# Autodesk Inventor assembly: 2 Falcon Single Reduction (WCP-0234)
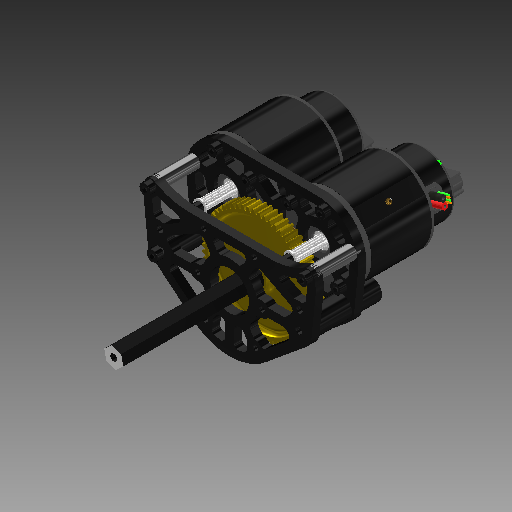
[picture p0: Inventor's stored thumbnail of the model, 512x512]
Saved by Autodesk Inventor 2023 (Build 270158000, 158)
## iProperties
Created: 2019-12-21
Part Number: 2 Falcon Single Reduction (WCP-0234)
Description: STEP AP214
Document SubType Name: Assembly
Designer: Desktop
Sending System: SolidWorks 2018
Preprocessor: SwSTEP 2.0
Title: WCP-0234 Rev1 - WCP SS Gearbox (Single Speed, 1 Stage).STEP
Revision Number: ANY
## iProperties of the stored document MemberDocs/xLqvepmqnB0sscau4Ttppawfh5h
Created: 2019-12-21
Part Number: 2 Falcon Single Reduction (WCP-0234)
Description: STEP AP214
Document SubType Name: Assembly
Designer: Desktop
Sending System: SolidWorks 2018
Preprocessor: SwSTEP 2.0
Title: WCP-0234 Rev1 - WCP SS Gearbox (Single Speed, 1 Stage).STEP
Revision Number: ANY
## iProperties of the stored document MemberDocs/x1zyynaqtFcftaj5mKokjps2x2f
Created: 2019-12-21
Part Number: 2 Falcon Single Reduction (WCP-0234)
Description: STEP AP214
Document SubType Name: Assembly
Designer: Desktop
Sending System: SolidWorks 2018
Preprocessor: SwSTEP 2.0
Title: WCP-0234 Rev1 - WCP SS Gearbox (Single Speed, 1 Stage).STEP
Revision Number: ANY
## iProperties of the stored document MemberDocs/xMxjli5cnGc0axyes40ohqydbMd
Created: 2019-12-21
Part Number: 2 Falcon Single Reduction (WCP-0234)
Description: STEP AP214
Document SubType Name: Assembly
Designer: Desktop
Sending System: SolidWorks 2018
Preprocessor: SwSTEP 2.0
Title: WCP-0234 Rev1 - WCP SS Gearbox (Single Speed, 1 Stage).STEP
Revision Number: ANY
## iProperties of the stored document MemberDocs/xPnixdcmtAsxrbsslCladjitsFg
Created: 2019-12-21
Part Number: 2 Falcon Single Reduction (WCP-0234)
Description: STEP AP214
Document SubType Name: Assembly
Designer: Desktop
Sending System: SolidWorks 2018
Preprocessor: SwSTEP 2.0
Title: WCP-0234 Rev1 - WCP SS Gearbox (Single Speed, 1 Stage).STEP
Revision Number: ANY
## Documents named in this file (62)
- C:\Users\Cal\Desktop\Robotics\Design\Collaborative\Collaborative Parts Library\Drivetrains\COTS WCD Gearboxes\2 Falcon Single Reduction (WCP-0234).iam
- C:\Users\Cal\Desktop\Robotics\Design\Collaborative\Collaborative Parts Library\Drivetrains\COTS WCD Gearboxes\2 Falcon Single Reduction (WCP-0234)\WCP-0234-001 Rev1.ipt
- C:\Users\Cal\Desktop\Robotics\Design\Collaborative\Collaborative Parts Library\Drivetrains\COTS WCD Gearboxes\2 Falcon Single Reduction (WCP-0234)\WCP-0234-002 Rev1.ipt
- C:\Users\Cal\Desktop\Robotics\Design\Collaborative\Collaborative Parts Library\Drivetrains\VersaChassis Parts\217-3437.ipt
- C:\Users\Cal\Desktop\Robotics\Design\Collaborative\Collaborative Parts Library\Power Transfer\Bearings and Bushings\Bearings\FR8 Hex.ipt
- E:\Middleton Robotics\Collaborative Robots\Collaborative Part Library\Power Transfer\Bearings.ipt
- C:\Users\Cal\Desktop\Robotics\Design\Collaborative\Collaborative Parts Library\Shaft Retention\Snaprings\Snapring for 0.5in Shaft (0.461in).ipt
- E:\Middleton Robotics\Collaborative Robots\Collaborative Part Library\Shaft Retention\Snaprings.ipt
- E:\Middleton Robotics\Collaborative Robots\Collaborative Part Library\Hardware\Machine Screws.ipt
- C:\Users\Cal\Desktop\Robotics\Design\Collaborative\Collaborative Parts Library\Hardware\Fasteners\Machine Screws\10-32 UNFx0.75 Socket Head Cap Screw.ipt
- E:\Middleton Robotics\Collaborative Robots\Collaborative Part Library\Hardware\Nuts.ipt
- C:\Users\Cal\Desktop\Robotics\Design\Collaborative\Collaborative Parts Library\Hardware\Nuts and Threaded Blocks\Nuts\10-32 Pan Head Nylon locknut.ipt
- C:\Users\Cal\Desktop\Robotics\Design\Collaborative\Collaborative Parts Library\Hardware\Fasteners\Machine Screws\10-32 UNFx0.25 Button Head Cap Screw.ipt
- C:\Users\Cal\Desktop\Robotics\Design\Collaborative\Collaborative Parts Library\Motors\FRC\Falcon 500.ipt
- C:\Users\Cal\Desktop\Robotics\Design\Collaborative\Collaborative Parts Library\Drivetrains\COTS WCD Gearboxes\2 Falcon Single Reduction (WCP-0234)\WCP-0234-003 Rev1.ipt
- C:\Users\Cal\Desktop\Robotics\Design\Collaborative\Collaborative Parts Library\Hardware\Fasteners\Machine Screws.ipt
- C:\Users\Cal\Desktop\Robotics\Design\Collaborative\Collaborative Parts Library\Hardware\Spacers\Spacers & Standoffs.ipt
- C:\Users\Cal\Desktop\Robotics\Design\Collaborative\Collaborative Parts Library\Hardware\Spacers\Spacers & Standoffs\WCP Aluminum Standoff (No. 10 x 1Lg x 0.375OD).ipt
- C:\Users\Cal\Desktop\Robotics\Design\Collaborative\Collaborative Parts Library\Hardware\Spacers\Spacers & Standoffs\Nylon Unthreaded Spacer (No. 10 x 1.25Lg x 0.625OD).ipt
- C:\Users\Cal\Desktop\Robotics\Design\Collaborative\Collaborative Parts Library\Motors\FRC\Motor Pinions.ipt
- C:\Users\Cal\Desktop\Robotics\Design\Collaborative\Collaborative Parts Library\Hardware\Fasteners\Machine Screws\8-32 UNCx0.25 Socket Head Cap Screw.ipt
- C:\Users\Cal\Desktop\Robotics\Design\Collaborative\Collaborative Parts Library\Hardware\Fasteners\Washers\Washer 0.174ID 0.375OD 0.038Thick.ipt
- E:\Middleton Robotics\Collaborative Robots\Collaborative Part Library\Hardware\Fasteners\Washers.ipt
- C:\Users\Cal\Desktop\Robotics\Design\Collaborative\Collaborative Parts Library\Power Transfer\Gears (Hex)\VexPro Spur Gears.ipt
- C:\Users\Cal\Desktop\Robotics\Design\Collaborative\Collaborative Parts Library\Hardware\Fasteners\Machine Screws\10-32 UNFx1.75 Socket Head Cap Screw.ipt
- C:\Users\Cal\Desktop\Robotics\Design\Collaborative\Collaborative Parts Library\Hardware\Fasteners\Machine Screws\10-32 UNFx2 Socket Head Cap Screw.ipt
- C:\Users\Cal\Desktop\Robotics\Design\Collaborative\Collaborative Parts Library\Power Transfer\Gears (Hex)\Spur Gear2\20dp 62T VexPro 500 Hex Aluminum Gear (Pocketed).ipt
- C:\Users\Cal\Desktop\Robotics\Design\Collaborative\Collaborative Parts Library\Hardware\Spacers\Spacers & Standoffs\WCP Aluminum Standoff (No. 10 x 1.25Lg x 0.375OD).ipt
- C:\Users\Cal\Desktop\Robotics\Design\Collaborative\Collaborative Parts Library\Hardware\Fasteners\Machine Screws\10-32 UNFx1.125 Socket Head Cap Screw.ipt
- E:\Middleton Robotics\Collaborative Robots\Collaborative Part Library\Drivetrains\COTS WCD Gearboxes\2 Falcon Single Reduction (WCP-0234)\WCP-0234-001 Rev1.ipt
- E:\Middleton Robotics\Collaborative Robots\Collaborative Part Library\Drivetrains\COTS WCD Gearboxes\2 Falcon Single Reduction (WCP-0234)\WCP-0234-002 Rev1.ipt
- E:\Middleton Robotics\Collaborative Robots\Collaborative Part Library\Drivetrains\217-3437.ipt
- E:\Middleton Robotics\Collaborative Robots\Collaborative Part Library\Power Transfer\Bearings and Bushings\Bearings\FR8 Hex.ipt
- E:\Middleton Robotics\Collaborative Robots\Collaborative Part Library\Shaft Retention\Snaprings\Snapring for 0.5in Shaft (0.461in).ipt
- E:\Middleton Robotics\Collaborative Robots\Collaborative Part Library\Hardware\Fasteners\Machine Screws\10-32 UNFx0.75 Socket Head Cap Screw.ipt
- E:\Middleton Robotics\Collaborative Robots\Collaborative Part Library\Hardware\Nuts and Threaded Blocks\Nuts\10-32 Pan Head Nylon locknut.ipt
- E:\Middleton Robotics\Collaborative Robots\Collaborative Part Library\Hardware\Fasteners\Machine Screws\10-32 UNFx0.25 Button Head Cap Screw.ipt
- E:\Middleton Robotics\Collaborative Robots\Collaborative Part Library\Motors\FRC\Falcon 500.ipt
- E:\Middleton Robotics\Collaborative Robots\Collaborative Part Library\Drivetrains\COTS WCD Gearboxes\2 Falcon Single Reduction (WCP-0234)\WCP-0234-003 Rev1.ipt
- E:\Middleton Robotics\Collaborative Robots\Collaborative Part Library\Hardware\Fasteners\Machine Screws.ipt
- E:\Middleton Robotics\Collaborative Robots\Collaborative Part Library\Hardware\Spacers\Spacers & Standoffs.ipt
- E:\Middleton Robotics\Collaborative Robots\Collaborative Part Library\Hardware\Spacers\Spacers & Standoffs\WCP Aluminum Standoff (No. 10 x 1Lg x 0.375OD).ipt
- E:\Middleton Robotics\Collaborative Robots\Collaborative Part Library\Hardware\Spacers\Spacers & Standoffs\Nylon Unthreaded Spacer (No. 10 x 1.25Lg x 0.625OD).ipt
- E:\Middleton Robotics\Collaborative Robots\Collaborative Part Library\Motors\FRC\Motor Pinions.ipt
- E:\Middleton Robotics\Collaborative Robots\Collaborative Part Library\Hardware\Fasteners\Machine Screws\8-32 UNCx0.25 Socket Head Cap Screw.ipt
- E:\Middleton Robotics\Collaborative Robots\Collaborative Part Library\Hardware\Fasteners\Washers\Washer 0.174ID 0.375OD 0.038Thick.ipt
- E:\Middleton Robotics\Collaborative Robots\Collaborative Part Library\Power Transfer\Gears (Hex)\VexPro Spur Gears.ipt
- E:\Middleton Robotics\Collaborative Robots\Collaborative Part Library\Hardware\Fasteners\Machine Screws\10-32 UNFx1.75 Socket Head Cap Screw.ipt
- E:\Middleton Robotics\Collaborative Robots\Collaborative Part Library\Hardware\Fasteners\Machine Screws\10-32 UNFx2 Socket Head Cap Screw.ipt
- E:\Middleton Robotics\Collaborative Robots\Collaborative Part Library\Power Transfer\Gears (Hex)\Spur Gear2\20dp 62T VexPro 500 Hex Aluminum Gear (Pocketed).ipt
- E:\Middleton Robotics\Collaborative Robots\Collaborative Part Library\Power Transfer\Gears (Hex)\Spur Gear2\20dp 58T VexPro 500 Hex Aluminum Gear (Pocketed).ipt
- E:\Middleton Robotics\Collaborative Robots\Collaborative Part Library\Power Transfer\VexPro Spur Gears.ipt
- E:\Middleton Robotics\Collaborative Robots\Collaborative Part Library\Drivetrains\VersaWheel Configurator.iam
- E:\Middleton Robotics\Collaborative Robots\Collaborative Part Library\Power Transfer\Sprockets\VexPro Sprockets.ipt
- E:\Middleton Robotics\Collaborative Robots\Collaborative Part Library\Power Transfer\Bearing Blocks\VersaBlock V2 (217-6111).ipt
- E:\Middleton Robotics\Collaborative Robots\Collaborative Part Library\Hardware\Fasteners\Washers\Washer 0.265ID 0.688OD 0.055Thick.ipt
- E:\Middleton Robotics\Collaborative Robots\Collaborative Part Library\Hardware\Retention\Washers.ipt
- E:\Middleton Robotics\Collaborative Robots\Collaborative Part Library\Hardware\Fasteners\Machine Screws\1(_FS)4-20 UNCx0.5 Button Head Cap Screw.ipt
- E:\Middleton Robotics\Collaborative Robots\Collaborative Part Library\Hardware\Fasteners\Machine Screws\10-32 UNFx1.5 Socket Head Cap Screw.ipt
- E:\Middleton Robotics\Collaborative Robots\Collaborative Part Library\Power Transfer\Sprockets\Sprockets\VexPro 12T 35 Chain 500 Hex Bore Double Sprocket.ipt
- E:\Middleton Robotics\Collaborative Robots\Collaborative Part Library\Hardware\Spacers\Spacers & Standoffs\WCP Aluminum Standoff (No. 10 x 1.75Lg x 0.375OD).ipt
- E:\Middleton Robotics\Collaborative Robots\Collaborative Part Library\Hardware\Fasteners\Machine Screws\10-32 UNFx2.5 Socket Head Cap Screw.ipt
## Components (35 placed, 20 different names)
1. WCP-0234-001 Rev1_1 — Insert:3, Mate:1, Mate:2, Insert:17, Insert:18, Insert:19, Insert:20, Insert:21, Insert:22, Insert:23, Insert:24, Insert:25, Insert:26, Insert:27, Flush:1, Insert:45, Insert:48
2. WCP-0234-002 Rev1_2 — Insert:6, Insert:7, Insert:13, Insert:14, Insert:15, Insert:16, Insert:32, Insert:33, Flush:2, Insert:42, Insert:44, Flush:3
3. 20dp 62T VexPro 500 Hex Aluminum Gear (Pocketed):1 — Insert:5
4. 217-3437:1 — Insert:4, Insert:12, Mate:6
5. FR8 Hex:1 — Insert:3, Insert:4, Insert:5
6. WCP Aluminum Standoff (No. 10 x 1.25Lg x 0.375OD):5 — Insert:7, Mate:2
7. WCP Aluminum Standoff (No. 10 x 1.25Lg x 0.375OD):4 — Insert:6, Mate:1, Insert:45, Insert:48
8. Snapring for 0.5in Shaft (0.461in):1 — Insert:12
9. 10-32 UNFx2 Socket Head Cap Screw:23 — Insert:14
10. 10-32 UNFx2 Socket Head Cap Screw:22 — Insert:13
11. 10-32 UNFx1.125 Socket Head Cap Screw:19 — Insert:16
12. 10-32 UNFx1.75 Socket Head Cap Screw:21 — Insert:15
13. 10-32 UNFx0.75 Socket Head Cap Screw:5 — Insert:18
14. 10-32 UNFx0.75 Socket Head Cap Screw:6 — Insert:17, Mate:4
15. 10-32 UNFx0.75 Socket Head Cap Screw:7 — Insert:19
16. 10-32 UNFx0.75 Socket Head Cap Screw:8 — Insert:21
17. 10-32 UNFx0.75 Socket Head Cap Screw:9 — Insert:22
18. 10-32 UNFx0.75 Socket Head Cap Screw:10 — Insert:20, Mate:5
19. 10-32 Pan Head Nylon locknut:1 — Insert:23
20. 10-32 Pan Head Nylon locknut:3 — Insert:24
21. Falcon 500:1 — Insert:26, Mate:5, Insert:49, Insert:52
22. Falcon 500:2 — Insert:27, Mate:4, Insert:50, Insert:54
23. WCP-0234-003 Rev1:1 — Insert:33
24. WCP-0234-003 Rev1:2 — Insert:32
25. WCP Aluminum Standoff (No. 10 x 1Lg x 0.375OD):10 — Insert:42
26. Nylon Unthreaded Spacer (No. 10 x 1.25Lg x 0.625OD):12 — Insert:44
27. Motor Pinions:1 — Insert:49
28. Motor Pinions:2 — Insert:50
29. 8-32 UNCx0.25 Socket Head Cap Screw:32 — Insert:51
30. Washer 0.174ID 0.375OD 0.038Thick:2 — Insert:51, Insert:52
31. 8-32 UNCx0.25 Socket Head Cap Screw:36
32. Washer 0.174ID 0.375OD 0.038Thick:3 — Insert:54
33. 10-32 UNFx0.25 Button Head Cap Screw:11 — Insert:25
34. 10-32 UNFx0.25 Button Head Cap Screw:12
35. 10-32 UNFx0.25 Button Head Cap Screw:13
## Component patterns: (3 elements, first: 10-32 UNFx0.25 Button Head Cap Screw:11)
## Relationships (41: Insert 33, Mate 5, Flush 3)
- Insert:3: WCP-0234-001 Rev1_1 ↔ FR8 Hex:1
- Insert:4: 217-3437:1 ↔ FR8 Hex:1
- Insert:5: 20dp 62T VexPro 500 Hex Aluminum Gear (Pocketed):1 ↔ FR8 Hex:1
- Insert:6: WCP-0234-002 Rev1_2 ↔ WCP Aluminum Standoff (No. 10 x 1.25Lg x 0.375OD):4
- Insert:7: WCP-0234-002 Rev1_2 ↔ WCP Aluminum Standoff (No. 10 x 1.25Lg x 0.375OD):5
- Mate:1: WCP-0234-001 Rev1_1 ↔ WCP Aluminum Standoff (No. 10 x 1.25Lg x 0.375OD):4
- Mate:2: WCP-0234-001 Rev1_1 ↔ WCP Aluminum Standoff (No. 10 x 1.25Lg x 0.375OD):5
- Insert:12: 217-3437:1 ↔ Snapring for 0.5in Shaft (0.461in):1
- Insert:13: WCP-0234-002 Rev1_2 ↔ 10-32 UNFx2 Socket Head Cap Screw:22
- Insert:14: WCP-0234-002 Rev1_2 ↔ 10-32 UNFx2 Socket Head Cap Screw:23
- Insert:15 (1.5875 mm): WCP-0234-002 Rev1_2 ↔ 10-32 UNFx1.75 Socket Head Cap Screw:21
- Insert:16 (1.5875 mm): WCP-0234-002 Rev1_2 ↔ 10-32 UNFx1.125 Socket Head Cap Screw:19
- Insert:17: WCP-0234-001 Rev1_1 ↔ 10-32 UNFx0.75 Socket Head Cap Screw:6
- Insert:18: WCP-0234-001 Rev1_1 ↔ 10-32 UNFx0.75 Socket Head Cap Screw:5
- Insert:19: WCP-0234-001 Rev1_1 ↔ 10-32 UNFx0.75 Socket Head Cap Screw:7
- Insert:20: WCP-0234-001 Rev1_1 ↔ 10-32 UNFx0.75 Socket Head Cap Screw:10
- Insert:21: WCP-0234-001 Rev1_1 ↔ 10-32 UNFx0.75 Socket Head Cap Screw:8
- Insert:22: WCP-0234-001 Rev1_1 ↔ 10-32 UNFx0.75 Socket Head Cap Screw:9
- Insert:23: WCP-0234-001 Rev1_1 ↔ 10-32 Pan Head Nylon locknut:1
- Insert:24: WCP-0234-001 Rev1_1 ↔ 10-32 Pan Head Nylon locknut:3
- Insert:25 (1.5875 mm): WCP-0234-001 Rev1_1 ↔ 10-32 UNFx0.25 Button Head Cap Screw:11
- Insert:26: WCP-0234-001 Rev1_1 ↔ Falcon 500:1
- Insert:27: WCP-0234-001 Rev1_1 ↔ Falcon 500:2
- Mate:4: 10-32 UNFx0.75 Socket Head Cap Screw:6 ↔ Falcon 500:2
- Mate:5: 10-32 UNFx0.75 Socket Head Cap Screw:10 ↔ Falcon 500:1
- Insert:32: WCP-0234-002 Rev1_2 ↔ WCP-0234-003 Rev1:2
- Insert:33: WCP-0234-002 Rev1_2 ↔ WCP-0234-003 Rev1:1
- Mate:6: 217-3437:1
- Flush:1: WCP-0234-001 Rev1_1
- Flush:2: WCP-0234-002 Rev1_2
- Insert:42: WCP-0234-002 Rev1_2 ↔ WCP Aluminum Standoff (No. 10 x 1Lg x 0.375OD):10
- Insert:44: WCP-0234-002 Rev1_2 ↔ Nylon Unthreaded Spacer (No. 10 x 1.25Lg x 0.625OD):12
- Insert:45: WCP-0234-001 Rev1_1 ↔ WCP Aluminum Standoff (No. 10 x 1.25Lg x 0.375OD):4
- Insert:48: WCP-0234-001 Rev1_1 ↔ WCP Aluminum Standoff (No. 10 x 1.25Lg x 0.375OD):4
- Insert:49: Falcon 500:1 ↔ Motor Pinions:1
- Insert:50: Falcon 500:2 ↔ Motor Pinions:2
- Flush:3: WCP-0234-002 Rev1_2
- Insert:51: 8-32 UNCx0.25 Socket Head Cap Screw:32 ↔ Washer 0.174ID 0.375OD 0.038Thick:2
- Insert:52: Falcon 500:1 ↔ Washer 0.174ID 0.375OD 0.038Thick:2
- [Insert]: 8-32 UNCx0.25 Socket Head Cap Screw:36 ↔ Washer 0.174ID 0.375OD 0.038Thick:3
- Insert:54: Falcon 500:2 ↔ Washer 0.174ID 0.375OD 0.038Thick:3
## Named parameters: d76_d74 = 0 mm
